# Autodesk Inventor assembly: PA_assemb
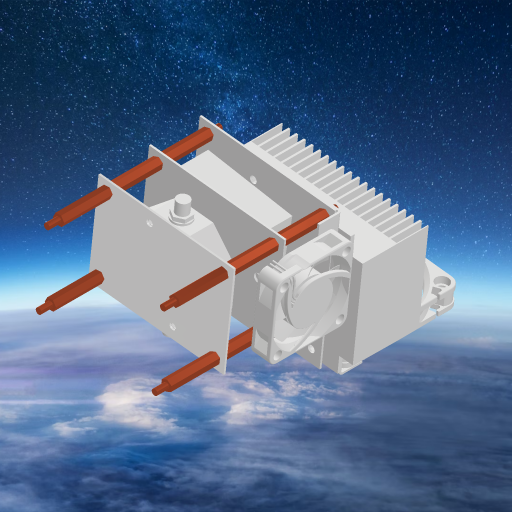
[picture p0: Inventor's stored thumbnail of the model, 512x512]
Saved by Autodesk Inventor 2023 (Build 270158000, 158)
## iProperties
Created: 2023-10-12
Part Number: PA_assemb
Document SubType Name: Assembly
Designer: 310611102
Author: 310611102
## Documents named in this file (12)
- C:\Users\310611102\Documents\Inventor\SSR\avionics_2023ver\assembly\PA_assemb.iam
- C:\Users\310611102\Documents\Inventor\SSR\avionics_2023ver\electronics\signal_combiner.ipt
- C:\Users\310611102\Documents\Inventor\SSR\avionics_2023ver\electronics\signal_combiner_plate.ipt
- C:\Users\310611102\Documents\Inventor\SSR\avionics_2023ver\electronics\copper_pillar_M3_L25.ipt
- C:\Users\310611102\Documents\Inventor\SSR\avionics_2023ver\electronics\power_amp_plate.ipt
- C:\Users\310611102\Documents\Inventor\SSR\avionics_2023ver\electronics\DCDCconvertor_plate.ipt
- C:\Users\310611102\Documents\Inventor\SSR\avionics_2023ver\electronics\DCDC24Vto15V.ipt
- C:\Users\310611102\Documents\Inventor\SSR\avionics_2023ver\electronics\EFB0612HA.ipt
- C:\Users\310611102\Documents\Inventor\SSR\avionics_2023ver\electronics\N0039 ERAM-0.01-1G-2W.ipt
- C:\Users\310611102\Documents\Inventor\SSR\avionics_2023ver\electronics\fan_fix_plate_connect.ipt
- C:\Users\310611102\Documents\Inventor\SSR\avionics_2023ver\electronics\fan_fix_plate_connect2.ipt
- C:\Users\310611102\Documents\Inventor\SSR\avionics_2023ver\electronics\CUI_DEVICES_CFM-4010V-150-157.ipt
## Components (22 placed, 11 different names)
1. signal_combiner:1
2. signal_combiner_plate:1 — Insert:27
3. copper_pillar_M3_L25:1
4. copper_pillar_M3_L25:2 — Insert:27
5. copper_pillar_M3_L25:3
6. copper_pillar_M3_L25:4
7. power_amp_plate:1 — Insert:28, Insert:29
8. DCDCconvertor_plate:1 — Insert:26
9. copper_pillar_M3_L25:5
10. copper_pillar_M3_L25:6
11. copper_pillar_M3_L25:7
12. copper_pillar_M3_L25:8
13. copper_pillar_M3_L25:9
14. copper_pillar_M3_L25:10
15. copper_pillar_M3_L25:11 — Insert:26
16. copper_pillar_M3_L25:12
17. DCDC24Vto15V:1
18. EFB0612HA:1
19. N0039 ERAM-0.01-1G-2W:1 — Insert:28, Insert:29
20. fan_fix_plate_connect:1
21. fan_fix_plate_connect2:1
22. CUI_DEVICES_CFM-4010V-150-157:1
## Relationships (31: Insert 29, Mate 1, Tangent 1)
- [Insert]: signal_combiner:1 ↔ signal_combiner_plate:1
- [Insert]: signal_combiner:1 ↔ signal_combiner_plate:1
- [Insert]: signal_combiner_plate:1 ↔ copper_pillar_M3_L25:1
- [Insert]: signal_combiner_plate:1 ↔ copper_pillar_M3_L25:4
- [Insert]: signal_combiner_plate:1 ↔ copper_pillar_M3_L25:3
- [Insert]: signal_combiner_plate:1 ↔ copper_pillar_M3_L25:5
- [Insert]: signal_combiner_plate:1 ↔ copper_pillar_M3_L25:6
- [Insert]: signal_combiner_plate:1 ↔ copper_pillar_M3_L25:7
- [Insert]: signal_combiner_plate:1 ↔ copper_pillar_M3_L25:8
- [Mate]: DCDCconvertor_plate:1 ↔ DCDC24Vto15V:1
- [Tangent]: DCDCconvertor_plate:1 ↔ DCDC24Vto15V:1
- [Insert]: DCDCconvertor_plate:1 ↔ copper_pillar_M3_L25:5
- [Insert]: DCDCconvertor_plate:1 ↔ copper_pillar_M3_L25:6
- [Insert]: DCDCconvertor_plate:1 ↔ copper_pillar_M3_L25:10
- [Insert]: DCDCconvertor_plate:1 ↔ copper_pillar_M3_L25:9
- [Insert]: DCDCconvertor_plate:1 ↔ copper_pillar_M3_L25:12
- [Insert]: EFB0612HA:1 ↔ fan_fix_plate_connect:1
- [Insert]: EFB0612HA:1 ↔ fan_fix_plate_connect:1
- [Insert]: power_amp_plate:1 ↔ copper_pillar_M3_L25:11
- [Insert]: power_amp_plate:1 ↔ copper_pillar_M3_L25:12
- [Insert]: power_amp_plate:1 ↔ N0039 ERAM-0.01-1G-2W:1
- [Insert]: N0039 ERAM-0.01-1G-2W:1 ↔ fan_fix_plate_connect:1
- [Insert]: N0039 ERAM-0.01-1G-2W:1 ↔ fan_fix_plate_connect:1
- [Insert]: power_amp_plate:1 ↔ fan_fix_plate_connect2:1
- [Insert]: power_amp_plate:1 ↔ fan_fix_plate_connect2:1
- [Insert]: fan_fix_plate_connect2:1 ↔ CUI_DEVICES_CFM-4010V-150-157:1
- [Insert]: fan_fix_plate_connect2:1 ↔ CUI_DEVICES_CFM-4010V-150-157:1
- Insert:26: DCDCconvertor_plate:1 ↔ copper_pillar_M3_L25:11
- Insert:27: signal_combiner_plate:1 ↔ copper_pillar_M3_L25:2
- Insert:28: power_amp_plate:1 ↔ N0039 ERAM-0.01-1G-2W:1
- Insert:29: power_amp_plate:1 ↔ N0039 ERAM-0.01-1G-2W:1
